# Autodesk Inventor assembly: side car
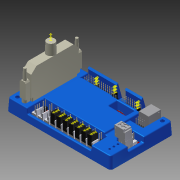
[picture p0: Inventor's stored thumbnail of the model, 180x180]
Saved by Autodesk Inventor 2013 (Build 170138000, 138)
## iProperties
Created: 2010-02-11
Part Number: side car
Document SubType Name: Assembly
Designer: Kyle
Author: Kyle
## Documents named in this file (5)
- \\lmss\STUDENTS\Robotics\CAD Files\COTS Parts\vkop\All-Electrical\side car.iam
- \\lmss\STUDENTS\Robotics\CAD Files\COTS Parts\vkop\All-Control-System\Control System_Diversified_Systems_A003333.ipt
- \\lmss\STUDENTS\Robotics\CAD Files\COTS Parts\vkop\All-Electrical\37 pin connector.ipt
- \\lmss\STUDENTS\Robotics\CAD Files\COTS Parts\vkop\All-Electrical\pwm connector.ipt
- \\lmss\STUDENTS\Robotics\CAD Files\COTS Parts\vkop\All-Electrical\pwm connector 3 pin.ipt
## Components (12 placed, 4 different names)
1. Control System_Diversified_Systems_A003333:1 — Mate:1, Mate:2, Mate:3, Mate:4, Mate:5, Flush:1, Mate:6, Mate:7, Mate:8, Mate:9, Flush:3, Mate:10, Mate:11, Mate:12, Mate:13, Flush:5, Mate:14, Mate:15, Mate:16, Mate:17, Mate:18, Mate:19, Mate:20, Mate:21, Mate:22, Mate:23, Mate:24, Mate:25, Mate:26
2. 37 pin connector:1 — Mate:1, Mate:2, Mate:3
3. pwm connector:1 — Mate:8, Mate:9, Flush:3, Flush:4
4. pwm connector:2 — Mate:12, Mate:13, Flush:5, Flush:6
5. pwm connector:3 — Mate:10, Mate:11, Flush:4
6. pwm connector:4 — Mate:6, Mate:7, Flush:2
7. pwm connector:5 — Mate:4, Mate:5, Flush:1, Flush:2
8. pwm connector:6 — Mate:16, Mate:17, Flush:7
9. pwm connector:7 — Mate:14, Mate:15, Flush:6, Flush:7
10. pwm connector 3 pin:1 — Mate:18, Mate:19, Mate:20
11. pwm connector 3 pin:2 — Mate:24, Mate:25, Mate:26
12. pwm connector 3 pin:3 — Mate:21, Mate:22, Mate:23
## Relationships (33: Mate 26, Flush 7)
- Mate:1: Control System_Diversified_Systems_A003333:1 ↔ 37 pin connector:1
- Mate:2: Control System_Diversified_Systems_A003333:1 ↔ 37 pin connector:1
- Mate:3: Control System_Diversified_Systems_A003333:1 ↔ 37 pin connector:1
- Mate:4: Control System_Diversified_Systems_A003333:1 ↔ pwm connector:5
- Mate:5: Control System_Diversified_Systems_A003333:1 ↔ pwm connector:5
- Flush:1: Control System_Diversified_Systems_A003333:1 ↔ pwm connector:5
- Mate:6: Control System_Diversified_Systems_A003333:1 ↔ pwm connector:4
- Mate:7: Control System_Diversified_Systems_A003333:1 ↔ pwm connector:4
- Flush:2: pwm connector:4 ↔ pwm connector:5
- Mate:8: Control System_Diversified_Systems_A003333:1 ↔ pwm connector:1
- Mate:9: Control System_Diversified_Systems_A003333:1 ↔ pwm connector:1
- Flush:3: Control System_Diversified_Systems_A003333:1 ↔ pwm connector:1
- Mate:10: Control System_Diversified_Systems_A003333:1 ↔ pwm connector:3
- Mate:11: Control System_Diversified_Systems_A003333:1 ↔ pwm connector:3
- Flush:4: pwm connector:1 ↔ pwm connector:3
- Mate:12: Control System_Diversified_Systems_A003333:1 ↔ pwm connector:2
- Mate:13: Control System_Diversified_Systems_A003333:1 ↔ pwm connector:2
- Flush:5: Control System_Diversified_Systems_A003333:1 ↔ pwm connector:2
- Mate:14: Control System_Diversified_Systems_A003333:1 ↔ pwm connector:7
- Mate:15: Control System_Diversified_Systems_A003333:1 ↔ pwm connector:7
- Flush:6: pwm connector:2 ↔ pwm connector:7
- Mate:16: Control System_Diversified_Systems_A003333:1 ↔ pwm connector:6
- Mate:17: Control System_Diversified_Systems_A003333:1 ↔ pwm connector:6
- Flush:7: pwm connector:6 ↔ pwm connector:7
- Mate:18: Control System_Diversified_Systems_A003333:1 ↔ pwm connector 3 pin:1
- Mate:19: Control System_Diversified_Systems_A003333:1 ↔ pwm connector 3 pin:1
- Mate:20: Control System_Diversified_Systems_A003333:1 ↔ pwm connector 3 pin:1
- Mate:21: Control System_Diversified_Systems_A003333:1 ↔ pwm connector 3 pin:3
- Mate:22: Control System_Diversified_Systems_A003333:1 ↔ pwm connector 3 pin:3
- Mate:23: Control System_Diversified_Systems_A003333:1 ↔ pwm connector 3 pin:3
- Mate:24: Control System_Diversified_Systems_A003333:1 ↔ pwm connector 3 pin:2
- Mate:25: Control System_Diversified_Systems_A003333:1 ↔ pwm connector 3 pin:2
- Mate:26: Control System_Diversified_Systems_A003333:1 ↔ pwm connector 3 pin:2
